# Autodesk Inventor assembly: A2017_T5_08
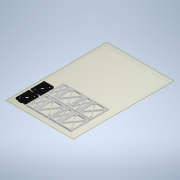
[picture p0: Inventor's stored thumbnail of the model, 180x180]
Saved by Autodesk Inventor 2020 (Build 240168000, 168)
## iProperties
Created: 2021-08-27
Part Number: A2017_T5_08
Document SubType Name: Assembly
Designer: Masato
Author: Masato
## Documents named in this file (5)
- D:\GitHub\inventor\SUSTAINA-OP\Cam\A2017_T5_08.iam
- D:\GitHub\inventor\SUSTAINA-OP\Cam\DisposableBoard.ipt
- D:\GitHub\inventor\SUSTAINA-OP\UpperBody\Arm\Shoulder_horn_frame.ipt
- D:\GitHub\inventor\SUSTAINA-OP\LowerBody\Link\BackLink_diagonal.ipt
- D:\GitHub\inventor\SUSTAINA-OP\LowerBody\Link\FrontLink_diagonal.ipt
## Components (11 placed, 4 different names)
1. DisposableBoard:1 — メイト:2, メイト:1, フラッシュ:1, フラッシュ:2, メイト:8, メイト:11, メイト:13, メイト:14, メイト:15, メイト:16, メイト:18
2. BackLink_diagonal:1 — メイト:14, メイト:15, メイト:17
3. FrontLink_diagonal:1 — メイト:13, メイト:16, メイト:17
4. BackLink_diagonal:2
5. FrontLink_diagonal:2
6. BackLink_diagonal:3
7. FrontLink_diagonal:3
8. BackLink_diagonal:4
9. FrontLink_diagonal:4
10. Shoulder_horn_frame:1 — メイト:8, メイト:11, メイト:18
11. Shoulder_horn_frame:2
## Component patterns: (4 elements, first: BackLink_diagonal:1 + FrontLink_diagonal:1), (2 elements, first: Shoulder_horn_frame:1)
## Relationships (12: Mate 10, Flush 2)
- メイト:2 [Mate]: DisposableBoard:1
- メイト:1 [Mate]: DisposableBoard:1
- フラッシュ:1 [Flush]: DisposableBoard:1
- フラッシュ:2 [Flush]: DisposableBoard:1
- メイト:8 [Mate]: DisposableBoard:1 ↔ Shoulder_horn_frame:1
- メイト:11 [Mate] (2 mm): DisposableBoard:1 ↔ Shoulder_horn_frame:1
- メイト:13 [Mate]: DisposableBoard:1 ↔ FrontLink_diagonal:1
- メイト:14 [Mate]: DisposableBoard:1 ↔ BackLink_diagonal:1
- メイト:15 [Mate] (2 mm): DisposableBoard:1 ↔ BackLink_diagonal:1
- メイト:16 [Mate] (2 mm): DisposableBoard:1 ↔ FrontLink_diagonal:1
- メイト:17 [Mate] (2.5 mm): BackLink_diagonal:1 ↔ FrontLink_diagonal:1
- メイト:18 [Mate] (2 mm): DisposableBoard:1 ↔ Shoulder_horn_frame:1
